# Autodesk Inventor assembly: Sensor Hoder and Sensor Assembly
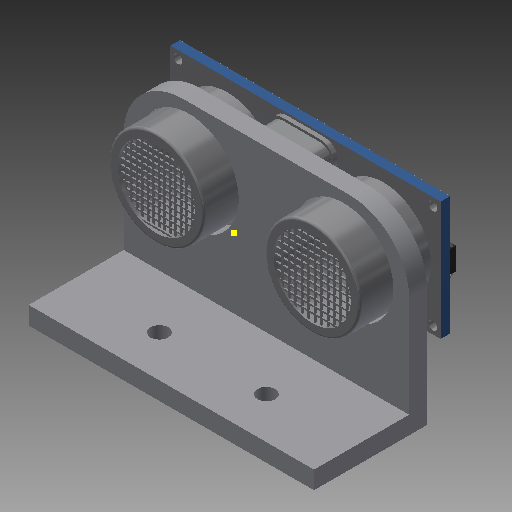
[picture p0: Inventor's stored thumbnail of the model, 512x512]
Saved by Autodesk Inventor 2017 (Build 210142000, 142)
## iProperties
Created: 2018-01-06
Part Number: Sensor Hoder and Sensor Assembly
Document SubType Name: Assembly
Designer: Dharsan
Author: Dharsan
## Documents named in this file (3)
- C:\Users\Dharsan\Desktop\Dharsan Innovation Files\Cart Model Inventor\Sensor Hoder and Sensor Assembly.iam
- C:\Users\Dharsan\Desktop\Dharsan Innovation Files\Cart Model Inventor\Ultrasonic Sensor Holder & Mount.ipt
- C:\Users\Dharsan\Desktop\Dharsan Innovation Files\Cart Model Inventor\Ultrasonic Sensor.ipt
## Components (2 placed, 2 different names)
1. Ultrasonic Sensor Holder & Mount:1 — Mate:1, Mate:2, Angle:1
2. Ultrasonic Sensor:1 — Mate:1, Mate:2, Angle:1
## Relationships (3: Mate 2, Angle 1)
- Mate:1: Ultrasonic Sensor Holder & Mount:1 ↔ Ultrasonic Sensor:1
- Mate:2: Ultrasonic Sensor Holder & Mount:1 ↔ Ultrasonic Sensor:1
- Angle:1 (180 deg): Ultrasonic Sensor Holder & Mount:1 ↔ Ultrasonic Sensor:1
